# Autodesk Inventor assembly: Optics Assembly Render
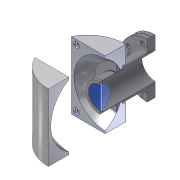
[picture p0: Inventor's stored thumbnail of the model, 180x180]
Saved by Autodesk Inventor 2015 SP1 (Build 190203100, 203)
## iProperties
Created: 2014-07-17
Part Number: Optics Assembly Render
Document SubType Name: Assembly
Designer: I Rabey
Author: I Rabey
## Documents named in this file (8)
- C:\ColdMatter\CADFiles\EDM Machine\Detection Region\Re-entrant Flange and Mirrors\Optics Assembly Render.iam
- C:\ColdMatter\CADFiles\EDM Machine\Detection Region\Re-entrant Flange and Mirrors\Mirrors\Ideas\Mirror Assembly.iam
- C:\ColdMatter\CADFiles\EDM Machine\Detection Region\Re-entrant Flange and Mirrors\Re-entrant Flange.iam
- C:\ColdMatter\CADFiles\EDM Machine\Detection Region\Re-entrant Flange and Mirrors\Mirrors\Custom Mirror Design.ipt
- C:\ColdMatter\CADFiles\EDM Machine\Detection Region\Re-entrant Flange and Mirrors\Mirrors\Custom Mirror Design Part 2.ipt
- C:\ColdMatter\CADFiles\EDM Machine\Detection Region\Re-entrant Flange and Mirrors\holdingRod.ipt
- C:\ColdMatter\CADFiles\EDM Machine\Detection Region\Re-entrant Flange and Mirrors\retainingring.ipt
- C:\ColdMatter\CADFiles\EDM Machine\Detection Region\Re-entrant Flange and Mirrors\scatterBlock.ipt
## Components (10 placed, 7 different names)
1. Mirror Assembly:1 [sub-assembly]
2. Re-entrant Flange:1 [sub-assembly] — Mate:20, Mate:21, Mate:25, Mate:30, Mate:33, Mate:35
3. Custom Mirror Design:1 — Mate:25, Mate:31, Mate:32
4. Custom Mirror Design Part 2:1 — Mate:21, Mate:27, Insert:1, Insert:2, Insert:3, Mate:29, Mate:30, Angle:1, Mate:32, Mate:34
5. holdingRod:1 — Insert:3
6. holdingRod:2 — Insert:1, Mate:31
7. holdingRod:3 — Insert:2
8. holdingRod:4 — Mate:29
9. retainingring:1 — Mate:33, Mate:34
10. scatterBlock:1 — Mate:35, Mate:36
## Relationships (18: Mate 14, Insert 3, Angle 1)
- Mate:11
- Mate:12
- Mate:20: Re-entrant Flange:1
- Mate:21: Re-entrant Flange:1 ↔ Custom Mirror Design Part 2:1
- Mate:25: Re-entrant Flange:1 ↔ Custom Mirror Design:1
- Mate:27 (75 mm): Custom Mirror Design Part 2:1
- Insert:1: Custom Mirror Design Part 2:1 ↔ holdingRod:2
- Insert:2: Custom Mirror Design Part 2:1 ↔ holdingRod:3
- Insert:3: Custom Mirror Design Part 2:1 ↔ holdingRod:1
- Mate:29: Custom Mirror Design Part 2:1 ↔ holdingRod:4
- Mate:30: Re-entrant Flange:1 ↔ Custom Mirror Design Part 2:1
- Mate:31: Custom Mirror Design:1 ↔ holdingRod:2
- Angle:1 (0 deg): Custom Mirror Design Part 2:1
- Mate:32 (75.75 mm): Custom Mirror Design:1 ↔ Custom Mirror Design Part 2:1
- Mate:33: Re-entrant Flange:1 ↔ retainingring:1
- Mate:34: Custom Mirror Design Part 2:1 ↔ retainingring:1
- Mate:35: Re-entrant Flange:1 ↔ scatterBlock:1
- Mate:36: scatterBlock:1
